# Autodesk Inventor assembly: 000 Ensamblaje hw_DAA - PCB FPGA
(part 2 of 2)
- Coincidencia:206 [Mate]: hw_DAA - PCB FPGA:1 ↔ GRT155R61E105KE01D:81
- Coincidencia:207 [Mate]: hw_DAA - PCB FPGA:1 ↔ GRT155C81C225KE13D:7
- Coincidencia:208 [Mate]: hw_DAA - PCB FPGA:1 ↔ GRT155R61A475ME13D:15
- Coincidencia:209 [Mate]: hw_DAA - PCB FPGA:1 ↔ GRT155R61A475ME13D:16
- Coincidencia:210 [Mate]: hw_DAA - PCB FPGA:1 ↔ CGA2B3X7R1H104K050BD:25
- Coincidencia:211 [Mate]: hw_DAA - PCB FPGA:1 ↔ CGA2B3X7R1H104K050BD:26
- Coincidencia:212 [Mate]: hw_DAA - PCB FPGA:1 ↔ GRT155R61E105KE01D:82
- Coincidencia:213 [Mate]: hw_DAA - PCB FPGA:1 ↔ GRT155C81C225KE13D:8
- Coincidencia:214 [Mate]: hw_DAA - PCB FPGA:1 ↔ CGA2B3X7R1H683K050BB:8
- Coincidencia:215 [Mate]: hw_DAA - PCB FPGA:1 ↔ CGA2B3X7R1H104K050BD:27
- Coincidencia:216 [Mate]: hw_DAA - PCB FPGA:1 ↔ GRT155R61A475ME13D:17
- Coincidencia:217 [Mate]: hw_DAA - PCB FPGA:1 ↔ GRT155R61A475ME13D:18
- Coincidencia:218 [Mate]: hw_DAA - PCB FPGA:1 ↔ GRT155R61A475ME13D:19
- Coincidencia:219 [Mate]: hw_DAA - PCB FPGA:1 ↔ GRT155R61E105KE01D:83
- Coincidencia:220 [Mate]: hw_DAA - PCB FPGA:1 ↔ GRT155R61E105KE01D:84
- Coincidencia:221 [Mate]: hw_DAA - PCB FPGA:1 ↔ GRM21BC80G107ME15L:16
- Coincidencia:222 [Mate]: hw_DAA - PCB FPGA:1 ↔ GRM21BC80G107ME15L:17
- Ángulo:14 [Angle] (0 deg): hw_DAA - PCB FPGA:1 ↔ GRM21BC80G107ME15L:16
- Ángulo:15 [Angle] (0 deg): hw_DAA - PCB FPGA:1 ↔ GRM21BC80G107ME15L:17
- Coincidencia:223 [Mate]: hw_DAA - PCB FPGA:1 ↔ GRT155R61E105KE01D:85
- Coincidencia:224 [Mate]: hw_DAA - PCB FPGA:1 ↔ GRT155R61E105KE01D:86
- Coincidencia:225 [Mate]: hw_DAA - PCB FPGA:1 ↔ GRT155R61A475ME13D:20
- Coincidencia:226 [Mate]: hw_DAA - PCB FPGA:1 ↔ GRT155R61A475ME13D:21
- Coincidencia:227 [Mate]: hw_DAA - PCB FPGA:1 ↔ CGA2B3X7R1H683K050BB:9
- Coincidencia:228 [Mate]: hw_DAA - PCB FPGA:1 ↔ GRT155R61A475ME13D:22
- Coincidencia:229 [Mate]: hw_DAA - PCB FPGA:1 ↔ CGA2B3X7R1H104K050BD:28
- Coincidencia:230 [Mate]: hw_DAA - PCB FPGA:1 ↔ GRT155C81C225KE13D:9
- Coincidencia:231 [Mate]: hw_DAA - PCB FPGA:1 ↔ GRT155R61E105KE01D:87
- Coincidencia:232 [Mate]: hw_DAA - PCB FPGA:1 ↔ CGA2B3X7R1H104K050BD:29
- Coincidencia:233 [Mate]: hw_DAA - PCB FPGA:1 ↔ CGA2B3X7R1H104K050BD:30
- Coincidencia:234 [Mate]: hw_DAA - PCB FPGA:1 ↔ GRT155R61A475ME13D:23
- Coincidencia:235 [Mate]: hw_DAA - PCB FPGA:1 ↔ GRT155R61A475ME13D:24
- Coincidencia:236 [Mate]: hw_DAA - PCB FPGA:1 ↔ GRT155C81C225KE13D:10
- Coincidencia:237 [Mate]: hw_DAA - PCB FPGA:1 ↔ GRT155R61E105KE01D:88
- Coincidencia:238 [Mate]: hw_DAA - PCB FPGA:1 ↔ CGA2B3X7R1H683K050BB:10
- Coincidencia:239 [Mate]: hw_DAA - PCB FPGA:1 ↔ CGA2B1X7S1C474K050BC:9
- Coincidencia:240 [Mate]: hw_DAA - PCB FPGA:1 ↔ CGA2B1X7S1C474K050BC:10
- Coincidencia:241 [Mate]: hw_DAA - PCB FPGA:1 ↔ CGA2B3X7R1H104K050BD:31
- Coincidencia:251 [Mate]: hw_DAA - PCB FPGA:1 ↔ CGA2B3X8R1H103K050BB:1
- Coincidencia:252 [Mate]: hw_DAA - PCB FPGA:1 ↔ GCM1555C1H101JA16D:1
- Coincidencia:253 [Mate]: hw_DAA - PCB FPGA:1 ↔ GRT155R61A475ME13D:25
- Coincidencia:254 [Mate]: hw_DAA - PCB FPGA:1 ↔ GRT155R61A475ME13D:26
- Coincidencia:255 [Mate]: hw_DAA - PCB FPGA:1 ↔ GRT155R61A475ME13D:27
- Ángulo:17 [Angle] (0 deg): hw_DAA - PCB FPGA:1 ↔ GRT155R61A475ME13D:25
- Ángulo:18 [Angle] (0 deg): hw_DAA - PCB FPGA:1 ↔ GRT155R61A475ME13D:26
- Ángulo:19 [Angle] (0 deg): hw_DAA - PCB FPGA:1 ↔ GRT155R61A475ME13D:27
- Coincidencia:256 [Mate]: hw_DAA - PCB FPGA:1 ↔ NFM18HC106D0G3L:2
- Coincidencia:257 [Mate]: hw_DAA - PCB FPGA:1 ↔ GRM21BC80G107ME15L:18
- Coincidencia:258 [Mate]: hw_DAA - PCB FPGA:1 ↔ GRT155D70G106ME13J:1
- Ángulo:20 [Angle] (0 deg): hw_DAA - PCB FPGA:1 ↔ GRT155D70G106ME13J:1
- Coincidencia:259 [Mate]: hw_DAA - PCB FPGA:1 ↔ GRT155D70G106ME13J:2
- Coincidencia:260 [Mate]: hw_DAA - PCB FPGA:1 ↔ CGA2B3X7R1H104K050BD:32
- Ángulo:21 [Angle] (0 deg): hw_DAA - PCB FPGA:1 ↔ CGA2B3X7R1H104K050BD:32
- Coincidencia:261 [Mate]: hw_DAA - PCB FPGA:1 ↔ GRT155D70G106ME13J:3
- Coincidencia:262 [Mate]: hw_DAA - PCB FPGA:1 ↔ GRT155D70G106ME13J:4
- Coincidencia:263 [Mate]: hw_DAA - PCB FPGA:1 ↔ NFM18HC106D0G3L:3
- Ángulo:22 [Angle] (0 deg): hw_DAA - PCB FPGA:1 ↔ NFM18HC106D0G3L:3
- Coincidencia:264 [Mate]: hw_DAA - PCB FPGA:1 ↔ GRT155D70G106ME13J:5
- Ángulo:23 [Angle] (0 deg): hw_DAA - PCB FPGA:1 ↔ GRT155D70G106ME13J:5
- Coincidencia:265 [Mate]: hw_DAA - PCB FPGA:1 ↔ CAPC-0603-T0.9-BN:1
- Ángulo:24 [Angle] (90 deg): hw_DAA - PCB FPGA:1 ↔ CAPC-0603-T0.9-BN:1
- Coincidencia:266 [Mate]: hw_DAA - PCB FPGA:1 ↔ GRT155R61A475ME13D:28
- Ángulo:25 [Angle] (0 deg): hw_DAA - PCB FPGA:1 ↔ GRT155R61A475ME13D:28
- Coincidencia:267 [Mate]: hw_DAA - PCB FPGA:1 ↔ GRT155R61A475ME13D:29
- Coincidencia:268 [Mate]: hw_DAA - PCB FPGA:1 ↔ GRT155R61A475ME13D:30
- Coincidencia:269 [Mate]: hw_DAA - PCB FPGA:1 ↔ ECS-.327-12.5-34QCS-TR:1
- Ángulo:26 [Angle] (0 deg): hw_DAA - PCB FPGA:1 ↔ ECS-.327-12.5-34QCS-TR:1
- Coincidencia:270 [Mate]: hw_DAA - PCB FPGA:1 ↔ SiT8008BI-11-33E-33.333333E:1
- Coincidencia:271 [Mate]: hw_DAA - PCB FPGA:1 ↔ CAPC-0603-T0.9-BN:2
- Coincidencia:272 [Mate]: hw_DAA - PCB FPGA:1 ↔ CAPC-0603-T0.9-BN:3
- Coincidencia:273 [Mate]: hw_DAA - PCB FPGA:1 ↔ CAPC-0603-T0.9-BN:4
- Coincidencia:274 [Mate]: hw_DAA - PCB FPGA:1 ↔ GRT155D70G106ME13J:6
- Coincidencia:275 [Mate]: hw_DAA - PCB FPGA:1 ↔ GRT155D70G106ME13J:7
- Coincidencia:276 [Mate]: hw_DAA - PCB FPGA:1 ↔ GRT155D70G106ME13J:8
- Coincidencia:277 [Mate]: hw_DAA - PCB FPGA:1 ↔ GRT155D70G106ME13J:9
- Coincidencia:278 [Mate]: hw_DAA - PCB FPGA:1 ↔ GRT155D70G106ME13J:10
- Ángulo:27 [Angle] (0 deg): hw_DAA - PCB FPGA:1 ↔ GRT155D70G106ME13J:10
- Coincidencia:279 [Mate]: hw_DAA - PCB FPGA:1 ↔ CGA2B3X7R1H104K050BD:33
- Ángulo:28 [Angle] (0 deg): hw_DAA - PCB FPGA:1 ↔ CGA2B3X7R1H104K050BD:33
- Coincidencia:280 [Mate]: hw_DAA - PCB FPGA:1 ↔ CGA2B1X7S1C474K050BC:11
- Ángulo:29 [Angle] (0 deg): hw_DAA - PCB FPGA:1 ↔ CGA2B1X7S1C474K050BC:11
- Coincidencia:281 [Mate]: hw_DAA - PCB FPGA:1 ↔ NFM18HC106D0G3L:4
- Ángulo:30 [Angle] (0 deg): hw_DAA - PCB FPGA:1 ↔ NFM18HC106D0G3L:4
- Coincidencia:282 [Mate]: hw_DAA - PCB FPGA:1 ↔ GRT155D70G106ME13J:11
- Ángulo:31 [Angle] (0 deg): hw_DAA - PCB FPGA:1 ↔ GRT155D70G106ME13J:11
- Coincidencia:283 [Mate]: hw_DAA - PCB FPGA:1 ↔ CAPC-0603-T0.9-BN:5
- Ángulo:32 [Angle] (0 deg): hw_DAA - PCB FPGA:1 ↔ CAPC-0603-T0.9-BN:5
- Coincidencia:284 [Mate]: hw_DAA - PCB FPGA:1 ↔ CAPC-0603-T0.9-BN:6
- Coincidencia:285 [Mate]: hw_DAA - PCB FPGA:1 ↔ GRT155D70G106ME13J:13
- Coincidencia:286 [Mate]: hw_DAA - PCB FPGA:1 ↔ GRT155D70G106ME13J:12
- Ángulo:33 [Angle] (0 deg): hw_DAA - PCB FPGA:1 ↔ GRT155D70G106ME13J:12
- Coincidencia:287 [Mate]: hw_DAA - PCB FPGA:1 ↔ GRT155D70G106ME13J:14
- Coincidencia:288 [Mate]: hw_DAA - PCB FPGA:1 ↔ GRT155D70G106ME13J:15
- Coincidencia:289 [Mate]: hw_DAA - PCB FPGA:1 ↔ GRT155D70G106ME13J:16
- Coincidencia:290 [Mate]: hw_DAA - PCB FPGA:1 ↔ GRT155D70G106ME13J:17
- Coincidencia:291 [Mate]: hw_DAA - PCB FPGA:1 ↔ GRT155D70G106ME13J:18
- Coincidencia:292 [Mate]: hw_DAA - PCB FPGA:1 ↔ GRT155D70G106ME13J:19
- Coincidencia:293 [Mate]: hw_DAA - PCB FPGA:1 ↔ 04025A220C4T2A:1
- Coincidencia:294 [Mate]: hw_DAA - PCB FPGA:1 ↔ CAPC-0402-T0.55-BN:1
- Coincidencia:295 [Mate]: hw_DAA - PCB FPGA:1 ↔ GRT155D70G106ME13J:20
- Ángulo:34 [Angle] (0 deg): hw_DAA - PCB FPGA:1 ↔ GRT155D70G106ME13J:20
- Coincidencia:296 [Mate]: hw_DAA - PCB FPGA:1 ↔ GRT155D70G106ME13J:21
- Ángulo:35 [Angle] (0 deg): hw_DAA - PCB FPGA:1 ↔ GRT155D70G106ME13J:21
- Coincidencia:297 [Mate]: hw_DAA - PCB FPGA:1 ↔ CGA2B3X7R1H104K050BD:34
- Ángulo:36 [Angle] (0 deg): hw_DAA - PCB FPGA:1 ↔ CGA2B3X7R1H104K050BD:34
- Coincidencia:298 [Mate]: hw_DAA - PCB FPGA:1 ↔ CGA2B1X7S1C474K050BC:12
- Ángulo:37 [Angle] (0 deg): hw_DAA - PCB FPGA:1 ↔ CGA2B1X7S1C474K050BC:12
- Coincidencia:299 [Mate]: hw_DAA - PCB FPGA:1 ↔ GRT155D70G106ME13J:22
- Coincidencia:300 [Mate]: hw_DAA - PCB FPGA:1 ↔ 04025A220C4T2A:2
- Ángulo:38 [Angle] (0 deg): hw_DAA - PCB FPGA:1 ↔ 04025A220C4T2A:2
- Coincidencia:301 [Mate]: hw_DAA - PCB FPGA:1 ↔ GRT155D70G106ME13J:23
- Coincidencia:302 [Mate]: hw_DAA - PCB FPGA:1 ↔ GRT155D70G106ME13J:24
- Ángulo:39 [Angle] (0 deg): hw_DAA - PCB FPGA:1 ↔ GRT155D70G106ME13J:24
- Coincidencia:303 [Mate]: hw_DAA - PCB FPGA:1 ↔ GRT155D70G106ME13J:25
- Coincidencia:304 [Mate]: hw_DAA - PCB FPGA:1 ↔ CAPC-0603-T0.9-BN:7
- Coincidencia:305 [Mate]: hw_DAA - PCB FPGA:1 ↔ TMP451HQDQFRQ1:1
- Coincidencia:306 [Mate]: hw_DAA - PCB FPGA:1 ↔ BZT52C3V3-7-F:1
- Coincidencia:307 [Mate]: hw_DAA - PCB FPGA:1 ↔ BZT52C3V3-7-F:1
- Coincidencia:314 [Mate]: hw_DAA - PCB FPGA:1 ↔ CRCW040239R0FKED:1
- Coincidencia:315 [Mate]: hw_DAA - PCB FPGA:1 ↔ CRCW040249R9FKED:1
- Coincidencia:316 [Mate]: hw_DAA - PCB FPGA:1 ↔ CRCW040249R9FKED:2
- Coincidencia:317 [Mate]: hw_DAA - PCB FPGA:1 ↔ CRCW040236R0FKED:1
- Coincidencia:318 [Mate]: hw_DAA - PCB FPGA:1 ↔ CRCW040236R0FKED:2
- Coincidencia:319 [Mate]: hw_DAA - PCB FPGA:1 ↔ ERJ-2GE0R00X:2
- Ángulo:40 [Angle] (0 deg): hw_DAA - PCB FPGA:1 ↔ ERJ-2GE0R00X:2
- Coincidencia:320 [Mate]: hw_DAA - PCB FPGA:1 ↔ ERJ-2RKF56R0X:2
- Coincidencia:321 [Mate]: hw_DAA - PCB FPGA:1 ↔ ERJ-2RKF56R0X:1
- Ángulo:41 [Angle] (0 deg): hw_DAA - PCB FPGA:1 ↔ ERJ-2RKF56R0X:1
- Ángulo:42 [Angle] (0 deg): hw_DAA - PCB FPGA:1 ↔ ERJ-2RKF56R0X:2
- Coincidencia:322 [Mate]: hw_DAA - PCB FPGA:1 ↔ ERJ-U02F4701X:9
- Coincidencia:323 [Mate]: hw_DAA - PCB FPGA:1 ↔ ERJ-U02F4701X:10
- Ángulo:43 [Angle] (0 deg): hw_DAA - PCB FPGA:1 ↔ ERJ-U02F4701X:9
- Ángulo:44 [Angle] (0 deg): hw_DAA - PCB FPGA:1 ↔ ERJ-U02F4701X:10
- Coincidencia:324 [Mate]: hw_DAA - PCB FPGA:1 ↔ CRCW0402240RFKED:1
- Coincidencia:325 [Mate]: hw_DAA - PCB FPGA:1 ↔ ERJ-U02F4701X:11
- Coincidencia:326 [Mate]: hw_DAA - PCB FPGA:1 ↔ ERJ-U02F4701X:12
- Coincidencia:327 [Mate]: hw_DAA - PCB FPGA:1 ↔ ERJ-U02F4701X:13
- Ángulo:45 [Angle] (0 deg): hw_DAA - PCB FPGA:1 ↔ ERJ-U02F4701X:12
- Ángulo:46 [Angle] (0 deg): hw_DAA - PCB FPGA:1 ↔ ERJ-U02F4701X:13
- Coincidencia:328 [Mate]: hw_DAA - PCB FPGA:1 ↔ CRCW0402240RFKED:2
- Coincidencia:329 [Mate]: hw_DAA - PCB FPGA:1 ↔ CRCW0402499RFKEDHP:1
- Coincidencia:330 [Mate]: hw_DAA - PCB FPGA:1 ↔ CRCW0402240RFKED:3
- Coincidencia:331 [Mate]: hw_DAA - PCB FPGA:1 ↔ CRCW0402499RFKEDHP:2
- Coincidencia:332 [Mate]: hw_DAA - PCB FPGA:1 ↔ CRCW0402240RFKED:4
- Coincidencia:333 [Mate]: hw_DAA - PCB FPGA:1 ↔ CRCW0402499RFKEDHP:3
- Ángulo:47 [Angle] (0 deg): hw_DAA - PCB FPGA:1 ↔ CRCW0402499RFKEDHP:3
- Coincidencia:334 [Mate]: hw_DAA - PCB FPGA:1 ↔ CRCW0402240RFKED:5
- Coincidencia:335 [Mate]: hw_DAA - PCB FPGA:1 ↔ CRCW0402499RFKEDHP:4
- Coincidencia:336 [Mate]: hw_DAA - PCB FPGA:1 ↔ CRCW0402240RFKED:6
- Coincidencia:337 [Mate]: hw_DAA - PCB FPGA:1 ↔ CRCW0402499RFKEDHP:5
- Coincidencia:338 [Mate]: hw_DAA - PCB FPGA:1 ↔ CRCW0402240RFKED:7
- Ángulo:48 [Angle] (90 deg): hw_DAA - PCB FPGA:1 ↔ CRCW0402240RFKED:7
- Coincidencia:339 [Mate]: hw_DAA - PCB FPGA:1 ↔ CRCW0402240RFKED:8
- Ángulo:49 [Angle] (0 deg): hw_DAA - PCB FPGA:1 ↔ CRCW0402240RFKED:8
- Coincidencia:340 [Mate]: hw_DAA - PCB FPGA:1 ↔ ERJ-2RKF1001X:1
- Coincidencia:341 [Mate]: hw_DAA - PCB FPGA:1 ↔ RC0402FR-7W100RL:1
- Ángulo:50 [Angle] (0 deg): hw_DAA - PCB FPGA:1 ↔ RC0402FR-7W100RL:1
- Coincidencia:342 [Mate]: hw_DAA - PCB FPGA:1 ↔ RC0402FR-7W100RL:2
- Coincidencia:343 [Mate]: hw_DAA - PCB FPGA:1 ↔ ERJ-2RKF1001X:2
- Coincidencia:344 [Mate]: hw_DAA - PCB FPGA:1 ↔ ERJ-2RKF1001X:3
- Ángulo:51 [Angle] (0 deg): hw_DAA - PCB FPGA:1 ↔ ERJ-2RKF1001X:3
- Coincidencia:345 [Mate]: hw_DAA - PCB FPGA:1 ↔ CRCW0402240RFKED:9
- Coincidencia:346 [Mate]: hw_DAA - PCB FPGA:1 ↔ CRCW0402240RFKED:10
- Coincidencia:347 [Mate]: hw_DAA - PCB FPGA:1 ↔ BLM15PX121SH1D:2
- Coincidencia:348 [Mate]: hw_DAA - PCB FPGA:1 ↔ BLM15PX121SH1D:1
- Ángulo:52 [Angle] (0 deg): hw_DAA - PCB FPGA:1 ↔ BLM15PX121SH1D:1
- Coincidencia:349 [Mate]: hw_DAA - PCB FPGA:1 ↔ ERJ-2RKF1001X:5
- Coincidencia:350 [Mate]: hw_DAA - PCB FPGA:1 ↔ ERJ-2RKF1001X:4
- Ángulo:53 [Angle] (0 deg): hw_DAA - PCB FPGA:1 ↔ ERJ-2RKF1001X:5
- Ángulo:54 [Angle] (0 deg): hw_DAA - PCB FPGA:1 ↔ ERJ-2RKF1001X:4
- Coincidencia:351 [Mate]: hw_DAA - PCB FPGA:1 ↔ RESC-0402:1
- Ángulo:55 [Angle] (0 deg): hw_DAA - PCB FPGA:1 ↔ RESC-0402:1
- Coincidencia:352 [Mate]: hw_DAA - PCB FPGA:1 ↔ ERJ-2RKF1001X:6
- Coincidencia:353 [Mate]: hw_DAA - PCB FPGA:1 ↔ RESC-0402:2
- Coincidencia:354 [Mate]: hw_DAA - PCB FPGA:1 ↔ CRCW0402240RFKED:11
- Ángulo:56 [Angle] (0 deg): hw_DAA - PCB FPGA:1 ↔ CRCW0402240RFKED:11
- Coincidencia:355 [Mate]: hw_DAA - PCB FPGA:1 ↔ ERJ-U02F4701X:14
- Ángulo:57 [Angle] (0 deg): hw_DAA - PCB FPGA:1 ↔ ERJ-U02F4701X:14
- Coincidencia:356 [Mate]: hw_DAA - PCB FPGA:1 ↔ CAPC-0603-T0.9-BN:8
- Ángulo:58 [Angle] (0 deg): hw_DAA - PCB FPGA:1 ↔ CAPC-0603-T0.9-BN:8
- Coincidencia:357 [Mate]: hw_DAA - PCB FPGA:1 ↔ CRCW0402499RFKEDHP:6
- Coincidencia:358 [Mate]: hw_DAA - PCB FPGA:1 ↔ CRCW0402499RFKEDHP:7
- Ángulo:59 [Angle] (0 deg): hw_DAA - PCB FPGA:1 ↔ CRCW0402499RFKEDHP:6
- Ángulo:60 [Angle] (0 deg): hw_DAA - PCB FPGA:1 ↔ CRCW0402499RFKEDHP:7
- Coincidencia:359 [Mate]: hw_DAA - PCB FPGA:1 ↔ ERJ-U02F4701X:15
- Ángulo:61 [Angle] (0 deg): hw_DAA - PCB FPGA:1 ↔ ERJ-U02F4701X:15
- Coincidencia:360 [Mate]: hw_DAA - PCB FPGA:1 ↔ ERJ-U02F4701X:16
- Coincidencia:361 [Mate]: hw_DAA - PCB FPGA:1 ↔ RESC-0402:3
- Ángulo:62 [Angle] (0 deg): hw_DAA - PCB FPGA:1 ↔ RESC-0402:3
- Coincidencia:362 [Mate]: hw_DAA - PCB FPGA:1 ↔ ERJ-U02F4701X:17
- Coincidencia:363 [Mate]: hw_DAA - PCB FPGA:1 ↔ ERJ-U02F4701X:18
- Ángulo:63 [Angle] (0 deg): hw_DAA - PCB FPGA:1 ↔ ERJ-U02F4701X:17
- Ángulo:64 [Angle] (0 deg): hw_DAA - PCB FPGA:1 ↔ ERJ-U02F4701X:18
- Coincidencia:364 [Mate]: hw_DAA - PCB FPGA:1 ↔ RESC-0402:4
- Ángulo:65 [Angle] (0 deg): hw_DAA - PCB FPGA:1 ↔ RESC-0402:4
- Coincidencia:365 [Mate]: hw_DAA - PCB FPGA:1 ↔ RESC-0402:5
- Ángulo:66 [Angle] (0 deg): hw_DAA - PCB FPGA:1 ↔ RESC-0402:5
- Coincidencia:366 [Mate]: hw_DAA - PCB FPGA:1 ↔ RESC-0402:6
- Coincidencia:367 [Mate]: hw_DAA - PCB FPGA:1 ↔ ERJ-U02F4701X:19
- Ángulo:67 [Angle] (0 deg): hw_DAA - PCB FPGA:1 ↔ ERJ-U02F4701X:19
- Coincidencia:368 [Mate]: hw_DAA - PCB FPGA:1 ↔ ERJ-U02F4701X:20
- Ángulo:68 [Angle] (0 deg): hw_DAA - PCB FPGA:1 ↔ ERJ-U02F4701X:20
- Coincidencia:369 [Mate]: hw_DAA - PCB FPGA:1 ↔ CRCW04024M70FKED:1
- Ángulo:69 [Angle] (0 deg): hw_DAA - PCB FPGA:1 ↔ CRCW04024M70FKED:1
- Coincidencia:370 [Mate]: hw_DAA - PCB FPGA:1 ↔ ERJ-U02F4701X:21
- Ángulo:70 [Angle] (0 deg): hw_DAA - PCB FPGA:1 ↔ ERJ-U02F4701X:21
- Coincidencia:371 [Mate]: hw_DAA - PCB FPGA:1 ↔ ERJ-2GE0R00X:3
- Coincidencia:372 [Mate]: hw_DAA - PCB FPGA:1 ↔ ERJ-U02F4701X:22
- Coincidencia:373 [Mate]: hw_DAA - PCB FPGA:1 ↔ RESC-0402:7
- Coincidencia:374 [Mate]: hw_DAA - PCB FPGA:1 ↔ RESC-0402:8
- Coincidencia:375 [Mate]: hw_DAA - PCB FPGA:1 ↔ ERJ-U02F4701X:23
- Coincidencia:376 [Mate]: hw_DAA - PCB FPGA:1 ↔ ERJ-U02F4701X:24
- Coincidencia:377 [Mate]: hw_DAA - PCB FPGA:1 ↔ RESC-0402:9
- Coincidencia:378 [Mate]: hw_DAA - PCB FPGA:1 ↔ ERJ-U02F4701X:25
- Coincidencia:379 [Mate]: hw_DAA - PCB FPGA:1 ↔ CRCW0402499RFKEDHP:8
- Ángulo:71 [Angle] (0 deg): hw_DAA - PCB FPGA:1 ↔ CRCW0402499RFKEDHP:8
- Coincidencia:380 [Mate]: hw_DAA - PCB FPGA:1 ↔ BLM15PX121SH1D:4
- Coincidencia:381 [Mate]: hw_DAA - PCB FPGA:1 ↔ BLM15PX121SH1D:3
- Ángulo:72 [Angle] (0 deg): hw_DAA - PCB FPGA:1 ↔ BLM15PX121SH1D:3
- Coincidencia:382 [Mate]: hw_DAA - PCB FPGA:1 ↔ CRCW0402240RFKED:12
- Ángulo:73 [Angle] (0 deg): hw_DAA - PCB FPGA:1 ↔ CRCW0402240RFKED:12
- [Mate]: hw_DAA - PCB FPGA:1 ↔ WP-SMRA Redcube (M2) 746630200:2
- Coincidencia:384 [Mate]: hw_DAA - PCB FPGA:1 ↔ WP-SMRA Redcube (M2) 7466302:2
- Ángulo:74 [Angle] (0 deg): hw_DAA - PCB FPGA:1 ↔ WP-SMRA Redcube (M2) 7466302:2
- Coincidencia:385 [Mate]: hw_DAA - PCB FPGA:1 ↔ WP-SMRA Redcube (M2) 7466302:3
- Ángulo:75 [Angle] (0 deg): hw_DAA - PCB FPGA:1 ↔ WP-SMRA Redcube (M2) 7466302:3
- [Mate]: hw_DAA - PCB FPGA:1 ↔ WP-SMRA Redcube (M2) 746630200:3
- Coincidencia:387 [Mate]: hw_DAA - PCB FPGA:1 ↔ WP-SMRA Redcube (M2) 746630200:1
- Ángulo:76 [Angle] (0 deg): hw_DAA - PCB FPGA:1 ↔ WP-SMRA Redcube (M2) 746630200:1
- Coincidencia:388 [Mate]: hw_DAA - PCB FPGA:1 ↔ CLP-106-02-F-D-BE-TR:2
- [Flush] (1.742 mm): hw_DAA - PCB FPGA:1 ↔ WP-SMRA Redcube (M2) 746630200:3
- Nivelación:2 [Flush]: hw_DAA - PCB FPGA:1 ↔ WP-SMRA Redcube (M2) 7466302:3
- Nivelación:3 [Flush]: hw_DAA - PCB FPGA:1 ↔ WP-SMRA Redcube (M2) 7466302:2
- [Flush] (1.742 mm): hw_DAA - PCB FPGA:1 ↔ WP-SMRA Redcube (M2) 746630200:2
- Ángulo:77 [Angle] (0 deg): hw_DAA - PCB FPGA:1 ↔ MT40A1G16TD-062E_AAT_F:5
- Ángulo:78 [Angle] (0 deg): hw_DAA - PCB FPGA:1 ↔ MT40A1G16TD-062E_AAT_F:4
- Ángulo:79 [Angle] (0 deg): hw_DAA - PCB FPGA:1 ↔ MT40A1G16TD-062E_AAT_F:3
- Ángulo:80 [Angle] (0 deg): hw_DAA - PCB FPGA:1 ↔ MT40A1G16TD-062E_AAT_F:2
- Ángulo:81 [Angle] (0 deg): hw_DAA - PCB FPGA:1 ↔ MT40A1G16TD-062E_AAT_F:1
- Ángulo:82 [Angle] (0 deg): hw_DAA - PCB FPGA:1 ↔ GRT155R61A475ME13D:29
- Ángulo:83 [Angle] (0 deg): hw_DAA - PCB FPGA:1 ↔ GRT155R61A475ME13D:30
- Ángulo:84 [Angle] (0 deg): hw_DAA - PCB FPGA:1 ↔ CGA2B3X8R1H103K050BB:1
- Ángulo:85 [Angle] (0 deg): hw_DAA - PCB FPGA:1 ↔ CRCW040249R9FKED:1
- Coincidencia:394 [Mate]: hw_DAA - PCB FPGA:1 ↔ CRCW040239R0FKED:2
- Coincidencia:395 [Mate]: hw_DAA - PCB FPGA:1 ↔ CRCW040239R0FKED:3
- Coincidencia:396 [Mate]: hw_DAA - PCB FPGA:1 ↔ CRCW040239R0FKED:4
- Coincidencia:397 [Mate]: hw_DAA - PCB FPGA:1 ↔ CRCW040239R0FKED:5
- Coincidencia:398 [Mate]: hw_DAA - PCB FPGA:1 ↔ CRCW040239R0FKED:6
- Coincidencia:399 [Mate]: hw_DAA - PCB FPGA:1 ↔ CRCW040239R0FKED:7
- Coincidencia:400 [Mate]: hw_DAA - PCB FPGA:1 ↔ CRCW040239R0FKED:8
- Coincidencia:401 [Mate]: hw_DAA - PCB FPGA:1 ↔ CRCW040239R0FKED:9
- Coincidencia:402 [Mate]: hw_DAA - PCB FPGA:1 ↔ CRCW040239R0FKED:10
- Coincidencia:403 [Mate]: hw_DAA - PCB FPGA:1 ↔ CRCW040239R0FKED:11
- Coincidencia:404 [Mate]: hw_DAA - PCB FPGA:1 ↔ CRCW040239R0FKED:12
- Coincidencia:405 [Mate]: hw_DAA - PCB FPGA:1 ↔ CRCW040239R0FKED:13
- Coincidencia:406 [Mate]: hw_DAA - PCB FPGA:1 ↔ CRCW040239R0FKED:14
- Coincidencia:407 [Mate]: hw_DAA - PCB FPGA:1 ↔ CRCW040239R0FKED:15
- Coincidencia:408 [Mate]: hw_DAA - PCB FPGA:1 ↔ CRCW040239R0FKED:16
- Coincidencia:409 [Mate]: hw_DAA - PCB FPGA:1 ↔ CRCW040239R0FKED:17
- Coincidencia:410 [Mate]: hw_DAA - PCB FPGA:1 ↔ CRCW040239R0FKED:18
- Coincidencia:411 [Mate]: hw_DAA - PCB FPGA:1 ↔ CRCW040239R0FKED:19
- Coincidencia:412 [Mate]: hw_DAA - PCB FPGA:1 ↔ CRCW040239R0FKED:20
- Coincidencia:413 [Mate]: hw_DAA - PCB FPGA:1 ↔ CRCW040239R0FKED:21
- Coincidencia:414 [Mate]: hw_DAA - PCB FPGA:1 ↔ CRCW040239R0FKED:22
- Coincidencia:415 [Mate]: hw_DAA - PCB FPGA:1 ↔ CRCW040239R0FKED:23
- Coincidencia:416 [Mate]: hw_DAA - PCB FPGA:1 ↔ CRCW040239R0FKED:24
- Coincidencia:417 [Mate]: hw_DAA - PCB FPGA:1 ↔ CRCW040239R0FKED:25
- Coincidencia:418 [Mate]: hw_DAA - PCB FPGA:1 ↔ GRT155R61E105KE01D:97
- Coincidencia:419 [Mate]: hw_DAA - PCB FPGA:1 ↔ GRT155R61E105KE01D:95
- Coincidencia:420 [Mate]: hw_DAA - PCB FPGA:1 ↔ GRT155R61E105KE01D:96
- Coincidencia:421 [Mate]: hw_DAA - PCB FPGA:1 ↔ GRT155R61E105KE01D:94
- Coincidencia:422 [Mate]: hw_DAA - PCB FPGA:1 ↔ GRT155R61E105KE01D:90
- Coincidencia:423 [Mate]: hw_DAA - PCB FPGA:1 ↔ GRT155R61E105KE01D:93
- Coincidencia:424 [Mate]: hw_DAA - PCB FPGA:1 ↔ GRT155R61E105KE01D:89
- Coincidencia:425 [Mate]: hw_DAA - PCB FPGA:1 ↔ GRT155R61E105KE01D:92
- Coincidencia:426 [Mate]: hw_DAA - PCB FPGA:1 ↔ GRT155R61E105KE01D:91
- Ángulo:86 [Angle] (0 deg): hw_DAA - PCB FPGA:1 ↔ GRT155R61E105KE01D:97
- [Mate] (-49.092 mm): hw_DAA - PCB FPGA:1 ↔ WP-SMRA Redcube (M2) 746630200:2
- Coincidencia:428 [Mate] (-12.01 mm): hw_DAA - PCB FPGA:1 ↔ WP-SMRA Redcube (M2) 7466302:3
- [Mate] (-45.1 mm): hw_DAA - PCB FPGA:1 ↔ WP-SMRA Redcube (M2) 746630200:3
- Nivelación:5 [Flush] (24.692 mm): hw_DAA - PCB FPGA:1 ↔ WP-SMRA Redcube (M2) 746630200:1
- Ángulo:87 [Angle] (0 deg): hw_DAA - PCB FPGA:1 ↔ CGA2B3X7R1H104K050BD:6
- Coincidencia:430 [Mate]: hw_DAA - PCB FPGA:1 ↔ ERJ-2RKF1001X:7
- Coincidencia:431 [Mate]: hw_DAA - PCB FPGA:1 ↔ ERJ-2RKF1002X:2
- Coincidencia:432 [Mate]: hw_DAA - PCB FPGA:1 ↔ ERJ-2RKF1002X:3
- Ángulo:88 [Angle] (0 deg): hw_DAA - PCB FPGA:1 ↔ ERJ-2RKF1002X:3
- Ángulo:89 [Angle] (0 deg): hw_DAA - PCB FPGA:1 ↔ ERJ-2RKF1002X:2
